# Autodesk Inventor assembly: baza
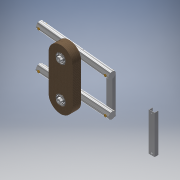
[picture p0: Inventor's stored thumbnail of the model, 180x180]
Saved by Autodesk Inventor 2017 (Build 210142000, 142)
## iProperties
Part Number: baza
Material: Ogólny
Document SubType Name: Assembly
Designer: Dorota
Author: Dorota
## Documents named in this file (6)
- F:\Dropbox\inventor\Rudder-Pedals\baza.iam
- F:\Dropbox\inventor\Rudder-Pedals\palak.iam
- F:\Dropbox\inventor\Rudder-Pedals\ceownik.ipt
- C:\Users\Golas\Documents\Inventor\Content Center Files\R2017\pl-PL\BS 290 SKF(29)\BS 290 SKF - SKF 6004-2RS1.ipt
- F:\Dropbox\inventor\Rudder-Pedals\tuleja-palak.ipt
- F:\Dropbox\inventor\Rudder-Pedals\podstawa.ipt
## Components (18 placed, 5 different names)
1. palak:1 [sub-assembly] — Równoległy:1, Obrotowe:6, Obrotowe:8, Obrotowe:9, Obrotowe:11, Obrotowe:13
2. palak:2 [sub-assembly] — Równoległy:1, Obrotowe:5, Obrotowe:7, Obrotowe:10, Obrotowe:12, Obrotowe:14
3. ceownik:1 — Równoległy:2
4. ceownik:2 — Równoległy:2
5. BS 290 SKF- z uszczelnieniem obustronnym SKF 6004-2RS1:1 — Obrotowe:5, Obrotowe:16
6. BS 290 SKF- z uszczelnieniem obustronnym SKF 6004-2RS1:2 — Obrotowe:6, Obrotowe:15
7. BS 290 SKF- z uszczelnieniem obustronnym SKF 6004-2RS1:3 — Obrotowe:18
8. BS 290 SKF- z uszczelnieniem obustronnym SKF 6004-2RS1:4 — Obrotowe:17
9. tuleja-palak:1 — Obrotowe:9
10. tuleja-palak:2 — Obrotowe:10
11. tuleja-palak:3 — Obrotowe:8
12. tuleja-palak:4 — Obrotowe:7
13. tuleja-palak:5 — Obrotowe:11
14. tuleja-palak:6 — Obrotowe:13
15. tuleja-palak:7 — Obrotowe:12
16. tuleja-palak:8 — Obrotowe:14
17. podstawa:1 — Zestawiający:1, Zestawiający:2, Zestawiający:3, Zestawiający:4, Obrotowe:17, Obrotowe:18, Zestawiający:5, Zestawiający:6
18. podstawa:2 — Zestawiający:1, Zestawiający:2, Zestawiający:3, Obrotowe:15, Obrotowe:16
## Relationships (22: RevoluteJoint 14, Mate 6, Flush 2)
- Równoległy:1 [Flush]: palak:1 ↔ palak:2
- Równoległy:2 [Flush]: ceownik:1 ↔ ceownik:2
- Obrotowe:5 [RevoluteJoint]: palak:2 ↔ BS 290 SKF- z uszczelnieniem obustronnym SKF 6004-2RS1:1
- Obrotowe:6 [RevoluteJoint]: palak:1 ↔ BS 290 SKF- z uszczelnieniem obustronnym SKF 6004-2RS1:2
- Obrotowe:7 [RevoluteJoint]: palak:2 ↔ tuleja-palak:4
- Obrotowe:8 [RevoluteJoint]: palak:1 ↔ tuleja-palak:3
- Obrotowe:9 [RevoluteJoint]: palak:1 ↔ tuleja-palak:1
- Obrotowe:10 [RevoluteJoint]: palak:2 ↔ tuleja-palak:2
- Obrotowe:11 [RevoluteJoint]: palak:1 ↔ tuleja-palak:5
- Obrotowe:12 [RevoluteJoint]: palak:2 ↔ tuleja-palak:7
- Obrotowe:13 [RevoluteJoint]: palak:1 ↔ tuleja-palak:6
- Obrotowe:14 [RevoluteJoint]: palak:2 ↔ tuleja-palak:8
- Zestawiający:1 [Mate]: podstawa:1 ↔ podstawa:2
- Zestawiający:2 [Mate]: podstawa:1 ↔ podstawa:2
- Zestawiający:3 [Mate]: podstawa:1 ↔ podstawa:2
- Zestawiający:4 [Mate]: podstawa:1
- Obrotowe:15 [RevoluteJoint]: BS 290 SKF- z uszczelnieniem obustronnym SKF 6004-2RS1:2 ↔ podstawa:2
- Obrotowe:16 [RevoluteJoint]: BS 290 SKF- z uszczelnieniem obustronnym SKF 6004-2RS1:1 ↔ podstawa:2
- Obrotowe:17 [RevoluteJoint]: BS 290 SKF- z uszczelnieniem obustronnym SKF 6004-2RS1:4 ↔ podstawa:1
- Obrotowe:18 [RevoluteJoint]: BS 290 SKF- z uszczelnieniem obustronnym SKF 6004-2RS1:3 ↔ podstawa:1
- Zestawiający:5 [Mate]: podstawa:1
- Zestawiający:6 [Mate]: podstawa:1
